# Autodesk Inventor assembly: 部件1
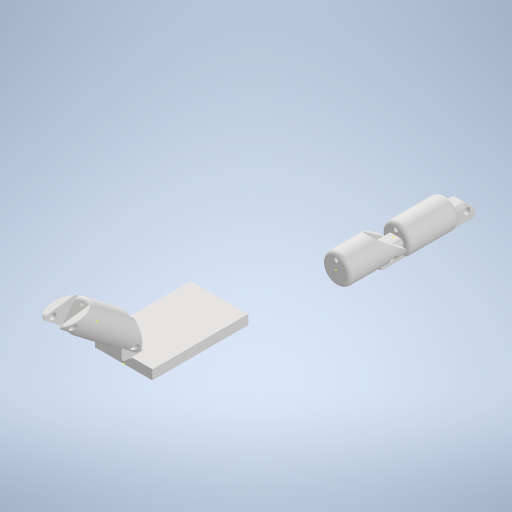
[picture p0: Inventor's stored thumbnail of the model, 512x512]
Saved by Autodesk Inventor 2023 (Build 270158000, 158)
## iProperties
Created: 2023-09-13
Part Number: 部件1
Document SubType Name: Assembly
Designer: Administrator
Author: Administrator
## Documents named in this file (5)
- C:\Users\Administrator\Desktop\部件1.iam
- C:\Users\Administrator\Desktop\零件1.ipt
- C:\Users\Administrator\Desktop\零件2.ipt
- C:\Users\Administrator\Desktop\零件3.ipt
- C:\Users\Administrator\Desktop\零件5.ipt
## Components (4 placed, 4 different names)
1. 零件1:1 — 配合:2, 配合:3
2. 零件2:1 — 配合:2, 配合:3
3. 零件3:1 — 配合:1, 配合:4, 配合:5
4. 零件5:1 — 配合:1, 配合:4, 配合:5
## Relationships (5: Mate 5)
- 配合:1 [Mate]: 零件3:1 ↔ 零件5:1
- 配合:2 [Mate]: 零件1:1 ↔ 零件2:1
- 配合:3 [Mate]: 零件1:1 ↔ 零件2:1
- 配合:4 [Mate]: 零件3:1 ↔ 零件5:1
- 配合:5 [Mate]: 零件3:1 ↔ 零件5:1
